# Autodesk Inventor assembly: UA-072 mit Denkmal
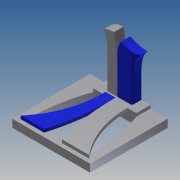
[picture p0: Inventor's stored thumbnail of the model, 180x180]
Saved by Autodesk Inventor 2015 (Build 190159000, 159)
## iProperties
Created: 2014-09-09
Part Number: UA-072 mit Denkmal
Document SubType Name: Assembly
Designer: Semenov
Author: Semenov
## Documents named in this file (6)
- W:\DATEN_INVENTOR\LiTHOS_FORMEN\UA\UA-072\UA-072 100x100\UA-072 mit Denkmal.iam
- W:\DATEN_INVENTOR\LiTHOS_FORMEN\UA\UA-072\UA-072 100x100\UA-072-EinfassungKT.ipt
- W:\DATEN_INVENTOR\LiTHOS_FORMEN\UA\UA-072\UA-072 100x100\UA-072-EinfassungST.ipt
- W:\DATEN_INVENTOR\LiTHOS_FORMEN\UA\UA-072\UA-072 100x100\UA-072-PlatteLinks.ipt
- W:\DATEN_INVENTOR\LiTHOS_FORMEN\UA\UA-072\UA-072 100x100\UA-072-PlatteRechts.ipt
- W:\DATEN_INVENTOR\LiTHOS_FORMEN\UA\UA-072\UA-072 100x100\UA-072-Denkmal.ipt
## Components (5 placed, 5 different names)
1. UA-072-EinfassungKT:1 — Passend:1, Passend:2, Fluchtend:1, Passend:3, Passend:4, Passend:5, Passend:6, Passend:7, Passend:8, Passend:9, Fluchtend:2, Fluchtend:3
2. UA-072-EinfassungST:1 — Passend:1, Passend:2, Fluchtend:1
3. UA-072-PlatteLinks:1 — Passend:3, Passend:4, Passend:5
4. UA-072-PlatteRechts:1 — Passend:6, Passend:7, Passend:8
5. UA-072-Denkmal:1 — Passend:9, Fluchtend:2, Fluchtend:3
## Relationships (12: Mate 9, Flush 3)
- Passend:1 [Mate]: UA-072-EinfassungKT:1 ↔ UA-072-EinfassungST:1
- Passend:2 [Mate]: UA-072-EinfassungKT:1 ↔ UA-072-EinfassungST:1
- Fluchtend:1 [Flush]: UA-072-EinfassungKT:1 ↔ UA-072-EinfassungST:1
- Passend:3 [Mate]: UA-072-EinfassungKT:1 ↔ UA-072-PlatteLinks:1
- Passend:4 [Mate]: UA-072-EinfassungKT:1 ↔ UA-072-PlatteLinks:1
- Passend:5 [Mate]: UA-072-EinfassungKT:1 ↔ UA-072-PlatteLinks:1
- Passend:6 [Mate]: UA-072-EinfassungKT:1 ↔ UA-072-PlatteRechts:1
- Passend:7 [Mate]: UA-072-EinfassungKT:1 ↔ UA-072-PlatteRechts:1
- Passend:8 [Mate]: UA-072-EinfassungKT:1 ↔ UA-072-PlatteRechts:1
- Passend:9 [Mate]: UA-072-EinfassungKT:1 ↔ UA-072-Denkmal:1
- Fluchtend:2 [Flush]: UA-072-EinfassungKT:1 ↔ UA-072-Denkmal:1
- Fluchtend:3 [Flush]: UA-072-EinfassungKT:1 ↔ UA-072-Denkmal:1
